# Autodesk Inventor assembly: robot_simplified
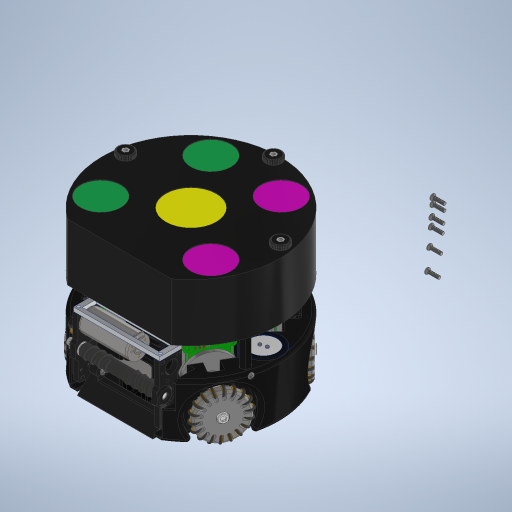
[picture p0: Inventor's stored thumbnail of the model, 512x512]
Saved by Autodesk Inventor 2023 (Build 270158000, 158)
## iProperties
Created: 2022-09-21
Part Number: robot_simplified
Document SubType Name: Assembly
Designer: victo
Author: victo
## Documents named in this file (19)
- C:\Users\victo\Documents\MATLAB\CAD\Inventor\robot_simplified.iam
- C:\Users\victo\Documents\MATLAB\CAD\Inventor\2021\Base_RoboCIn.ipt
- C:\Users\victo\Documents\MATLAB\CAD\Inventor\2021\SupportFirstToSecond.ipt
- C:\Users\victo\Documents\MATLAB\CAD\Inventor\2021\plate_sec_floor.ipt
- C:\Users\victo\Documents\MATLAB\CAD\Inventor\2021\SupportSecondToCoverNew.ipt
- C:\Users\victo\Documents\MATLAB\CAD\Inventor\2021\CoverNew.ipt
- C:\Users\victo\Documents\MATLAB\CAD\Inventor\2021\tag_green.ipt
- C:\Users\victo\Documents\MATLAB\CAD\Inventor\2021\tag_magenta.ipt
- C:\Users\victo\Documents\MATLAB\CAD\Inventor\2021\tag_yellow.ipt
- C:\Users\victo\Documents\MATLAB\CAD\Inventor\sec_floor\tampa_nut.ipt
- C:\Users\victo\Documents\MATLAB\CAD\Inventor\first_floor\Wheel\RoboCinWheel_simplified.iam
- C:\Users\victo\Documents\MATLAB\CAD\Inventor\first_floor\Kicker\kicker_assembly.iam
- C:\Users\victo\Documents\MATLAB\CAD\Inventor\first_floor\Motor\MaxonEC45-50W-MILE-Machined-with-gear.iam
- C:\Users\victo\Documents\MATLAB\CAD\Inventor\first_floor\Components\Battery4S.ipt
- C:\Users\victo\Documents\MATLAB\CAD\Inventor\first_floor\Components\Capacitor.ipt
- C:\Users\victo\Documents\MATLAB\CAD\Inventor\sec_floor\standoff.ipt
- C:\Users\victo\Documents\MATLAB\CAD\Inventor\sec_floor\standoffAdapter.ipt
- C:\Users\victo\Documents\MATLAB\CAD\Inventor\first_floor\Dribbler-3-gears\Dribbler-3-gears-new.iam
- C:\Users\victo\Documents\MATLAB\CAD\Inventor\other\m3-10mm.ipt
## Components (56 placed, 18 different names)
1. Base_RoboCIn:1 — Mate:1, Mate:2, Mate:3, Mate:4, Mate:5, Mate:6, Mate:7, Mate:8, Coincidente:9, Ângulo:1, Coincidente:10, Coincidente:11, Coincidente:12, Coincidente:13, Coincidente:14, Coincidente:15, Coincidente:16, Coincidente:17, Coincidente:18, Coincidente:19, Coincidente:20, Coincidente:21, Coincidente:22, Coincidente:23, Coincidente:24, Coincidente:25, Coincidente:26, Coincidente:27, Coincidente:28, Coincidente:29, Coincidente:42, Coincidente:43, Ângulo:5, Coincidente:44, Coincidente:45, Coincidente:46, Coincidente:47, Coincidente:48, Coincidente:50, Coincidente:51, Coincidente:52, Coincidente:71, Coincidente:72, Coincidente:75, Coincidente:76
2. SupportFirstToSecond:1
3. SupportFirstToSecond:2
4. SupportFirstToSecond:3
5. SupportFirstToSecond:4
6. plate_sec_floor:1
7. SupportSecondToCoverNew:1
8. SupportSecondToCoverNew:2
9. CoverNew:1 — Coincidente:30, Coincidente:32, Coincidente:33, Coincidente:34, Coincidente:35, Coincidente:39, Coincidente:40, Coincidente:41
10. tag_green:1
11. tag_green:2
12. tag_magenta:1
13. tag_magenta:2
14. tag_yellow:1
15. tampa_nut:1 — Coincidente:31
16. RoboCinWheel_simplified:1 [sub-assembly] — Mate:1, Mate:5
17. RoboCinWheel_simplified:2 [sub-assembly] — Mate:2, Mate:6
18. RoboCinWheel_simplified:3 [sub-assembly] — Mate:3, Mate:8
19. RoboCinWheel_simplified:4 [sub-assembly] — Mate:4, Mate:7
20. Kicker Assembly:1 [sub-assembly] — Coincidente:9, Ângulo:1, Coincidente:10, Coincidente:53, Coincidente:54, Coincidente:55, Coincidente:56, Coincidente:57, Coincidente:58, Coincidente:59, Coincidente:60, Coincidente:62, Coincidente:63, Coincidente:64, Coincidente:65, Coincidente:66, Coincidente:67, Coincidente:68
21. MG-MaxonEC45-50W-MILE:1 [sub-assembly] — Coincidente:17, Coincidente:18, Coincidente:19
22. MG-MaxonEC45-50W-MILE:2 [sub-assembly] — Coincidente:11, Coincidente:12, Coincidente:13
23. MG-MaxonEC45-50W-MILE:3 [sub-assembly] — Coincidente:14, Coincidente:15, Coincidente:16
24. MG-MaxonEC45-50W-MILE:4 [sub-assembly] — Coincidente:20, Coincidente:21, Coincidente:22
25. Battery4S:1 — Coincidente:23, Coincidente:24, Coincidente:25
26. Capacitor:1 — Coincidente:27, Coincidente:28
27. Capacitor:2 — Coincidente:26, Coincidente:29
28. standoff:1 — Coincidente:30, Coincidente:35, Coincidente:37, Ângulo:3
29. standoff:2 — Coincidente:31, Coincidente:34, Coincidente:38, Ângulo:2
30. standoff:3 — Coincidente:32, Coincidente:33, Coincidente:36, Ângulo:4
31. standoffAdapter:1 — Coincidente:37, Ângulo:3, Coincidente:41
32. standoffAdapter:2 — Coincidente:38, Ângulo:2, Coincidente:40
33. standoffAdapter:3 — Coincidente:36, Ângulo:4, Coincidente:39
34. Dribbler-3-gears-new:1 [sub-assembly] — Coincidente:42, Coincidente:43, Ângulo:5, Coincidente:69, Coincidente:70, Coincidente:73, Coincidente:74
35. m3-10mm:1 — Coincidente:44, Coincidente:52
36. m3-10mm:2 — Coincidente:45, Coincidente:50
37. m3-10mm:3 — Coincidente:47, Coincidente:48
38. m3-10mm:4 — Coincidente:46, Coincidente:51
39. m3-10mm:5 — Coincidente:53, Coincidente:67
40. m3-10mm:6 — Coincidente:54, Coincidente:64
41. m3-10mm:7 — Coincidente:55
42. m3-10mm:8 — Coincidente:57, Coincidente:63
43. m3-10mm:9 — Coincidente:56, Coincidente:65
44. m3-10mm:10 — Coincidente:58, Coincidente:62
45. m3-10mm:11 — Coincidente:59, Coincidente:66
46. m3-10mm:12 — Coincidente:60, Coincidente:68
47. m3-10mm:13 — Coincidente:69, Coincidente:73
48. m3-10mm:14 — Coincidente:70, Coincidente:74
49. m3-10mm:15 — Coincidente:71, Coincidente:75
50. m3-10mm:16 — Coincidente:72, Coincidente:76
51. m3-10mm:17
52. m3-10mm:18
53. m3-10mm:19
54. m3-10mm:20
55. m3-10mm:21
56. m3-10mm:22
## Relationships (79: Mate 74, Angle 5)
- Mate:1: Base_RoboCIn:1 ↔ RoboCinWheel_simplified:1
- Mate:2: Base_RoboCIn:1 ↔ RoboCinWheel_simplified:2
- Mate:3: Base_RoboCIn:1 ↔ RoboCinWheel_simplified:3
- Mate:4: Base_RoboCIn:1 ↔ RoboCinWheel_simplified:4
- Mate:5 (1 mm): Base_RoboCIn:1 ↔ RoboCinWheel_simplified:1
- Mate:6 (1 mm): Base_RoboCIn:1 ↔ RoboCinWheel_simplified:2
- Mate:7 (1 mm): Base_RoboCIn:1 ↔ RoboCinWheel_simplified:4
- Mate:8 (1 mm): Base_RoboCIn:1 ↔ RoboCinWheel_simplified:3
- Coincidente:9 [Mate]: Base_RoboCIn:1 ↔ Kicker Assembly:1
- Ângulo:1 [Angle] (0 deg): Base_RoboCIn:1 ↔ Kicker Assembly:1
- Coincidente:10 [Mate]: Base_RoboCIn:1 ↔ Kicker Assembly:1
- Coincidente:11 [Mate]: Base_RoboCIn:1 ↔ MG-MaxonEC45-50W-MILE:2
- Coincidente:12 [Mate]: Base_RoboCIn:1 ↔ MG-MaxonEC45-50W-MILE:2
- Coincidente:13 [Mate]: Base_RoboCIn:1 ↔ MG-MaxonEC45-50W-MILE:2
- Coincidente:14 [Mate]: Base_RoboCIn:1 ↔ MG-MaxonEC45-50W-MILE:3
- Coincidente:15 [Mate]: Base_RoboCIn:1 ↔ MG-MaxonEC45-50W-MILE:3
- Coincidente:16 [Mate]: Base_RoboCIn:1 ↔ MG-MaxonEC45-50W-MILE:3
- Coincidente:17 [Mate]: Base_RoboCIn:1 ↔ MG-MaxonEC45-50W-MILE:1
- Coincidente:18 [Mate]: Base_RoboCIn:1 ↔ MG-MaxonEC45-50W-MILE:1
- Coincidente:19 [Mate]: Base_RoboCIn:1 ↔ MG-MaxonEC45-50W-MILE:1
- Coincidente:20 [Mate]: Base_RoboCIn:1 ↔ MG-MaxonEC45-50W-MILE:4
- Coincidente:21 [Mate]: Base_RoboCIn:1 ↔ MG-MaxonEC45-50W-MILE:4
- Coincidente:22 [Mate]: Base_RoboCIn:1 ↔ MG-MaxonEC45-50W-MILE:4
- Coincidente:23 [Mate]: Base_RoboCIn:1 ↔ Battery4S:1
- Coincidente:24 [Mate] (2 mm): Base_RoboCIn:1 ↔ Battery4S:1
- Coincidente:25 [Mate] (2 mm): Base_RoboCIn:1 ↔ Battery4S:1
- Coincidente:26 [Mate]: Base_RoboCIn:1 ↔ Capacitor:2
- Coincidente:27 [Mate]: Base_RoboCIn:1 ↔ Capacitor:1
- Coincidente:28 [Mate]: Base_RoboCIn:1 ↔ Capacitor:1
- Coincidente:29 [Mate]: Base_RoboCIn:1 ↔ Capacitor:2
- Coincidente:30 [Mate]: CoverNew:1 ↔ standoff:1
- Coincidente:31 [Mate]: tampa_nut:1 ↔ standoff:2
- Coincidente:32 [Mate]: CoverNew:1 ↔ standoff:3
- Coincidente:33 [Mate]: CoverNew:1 ↔ standoff:3
- Coincidente:34 [Mate]: CoverNew:1 ↔ standoff:2
- Coincidente:35 [Mate]: CoverNew:1 ↔ standoff:1
- Coincidente:36 [Mate]: standoff:3 ↔ standoffAdapter:3
- Coincidente:37 [Mate]: standoff:1 ↔ standoffAdapter:1
- Coincidente:38 [Mate]: standoff:2 ↔ standoffAdapter:2
- Ângulo:2 [Angle] (0 deg): standoff:2 ↔ standoffAdapter:2
- Ângulo:3 [Angle] (0 deg): standoff:1 ↔ standoffAdapter:1
- Ângulo:4 [Angle] (0 deg): standoff:3 ↔ standoffAdapter:3
- Coincidente:39 [Mate]: CoverNew:1 ↔ standoffAdapter:3
- Coincidente:40 [Mate]: CoverNew:1 ↔ standoffAdapter:2
- Coincidente:41 [Mate]: CoverNew:1 ↔ standoffAdapter:1
- Coincidente:42 [Mate]: Base_RoboCIn:1 ↔ Dribbler-3-gears-new:1
- Coincidente:43 [Mate] (2 mm): Base_RoboCIn:1 ↔ Dribbler-3-gears-new:1
- Ângulo:5 [Angle] (0 deg): Base_RoboCIn:1 ↔ Dribbler-3-gears-new:1
- Coincidente:44 [Mate]: Base_RoboCIn:1 ↔ m3-10mm:1
- Coincidente:45 [Mate]: Base_RoboCIn:1 ↔ m3-10mm:2
- Coincidente:46 [Mate]: Base_RoboCIn:1 ↔ m3-10mm:4
- Coincidente:47 [Mate]: Base_RoboCIn:1 ↔ m3-10mm:3
- Coincidente:48 [Mate]: Base_RoboCIn:1 ↔ m3-10mm:3
- Coincidente:50 [Mate]: Base_RoboCIn:1 ↔ m3-10mm:2
- Coincidente:51 [Mate]: Base_RoboCIn:1 ↔ m3-10mm:4
- Coincidente:52 [Mate]: Base_RoboCIn:1 ↔ m3-10mm:1
- Coincidente:53 [Mate]: Kicker Assembly:1 ↔ m3-10mm:5
- Coincidente:54 [Mate]: Kicker Assembly:1 ↔ m3-10mm:6
- Coincidente:55 [Mate]: Kicker Assembly:1 ↔ m3-10mm:7
- Coincidente:56 [Mate]: Kicker Assembly:1 ↔ m3-10mm:9
- Coincidente:57 [Mate]: Kicker Assembly:1 ↔ m3-10mm:8
- Coincidente:58 [Mate]: Kicker Assembly:1 ↔ m3-10mm:10
- Coincidente:59 [Mate]: Kicker Assembly:1 ↔ m3-10mm:11
- Coincidente:60 [Mate]: Kicker Assembly:1 ↔ m3-10mm:12
- Coincidente:62 [Mate]: Kicker Assembly:1 ↔ m3-10mm:10
- Coincidente:63 [Mate]: Kicker Assembly:1 ↔ m3-10mm:8
- Coincidente:64 [Mate]: Kicker Assembly:1 ↔ m3-10mm:6
- Coincidente:65 [Mate]: Kicker Assembly:1 ↔ m3-10mm:9
- Coincidente:66 [Mate]: Kicker Assembly:1 ↔ m3-10mm:11
- Coincidente:67 [Mate]: Kicker Assembly:1 ↔ m3-10mm:5
- Coincidente:68 [Mate]: Kicker Assembly:1 ↔ m3-10mm:12
- Coincidente:69 [Mate]: Dribbler-3-gears-new:1 ↔ m3-10mm:13
- Coincidente:70 [Mate]: Dribbler-3-gears-new:1 ↔ m3-10mm:14
- Coincidente:71 [Mate]: Base_RoboCIn:1 ↔ m3-10mm:15
- Coincidente:72 [Mate]: Base_RoboCIn:1 ↔ m3-10mm:16
- Coincidente:73 [Mate]: Dribbler-3-gears-new:1 ↔ m3-10mm:13
- Coincidente:74 [Mate]: Dribbler-3-gears-new:1 ↔ m3-10mm:14
- Coincidente:75 [Mate]: Base_RoboCIn:1 ↔ m3-10mm:15
- Coincidente:76 [Mate]: Base_RoboCIn:1 ↔ m3-10mm:16
